# Autodesk Inventor assembly: WheelAssembly
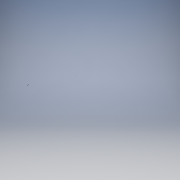
[picture p0: Inventor's stored thumbnail of the model, 180x180]
Saved by Autodesk Inventor 2016 (Build 200138000, 138)
## iProperties
Created: 2016-09-10
Part Number: WheelAssembly
Document SubType Name: Assembly
Designer: RoboticsUser
Author: RoboticsUser
## Documents named in this file (10)
- C:\Robotics\2016-17_CAD\WheelAssembly.iam
- C:\Robotics\CAD\2015-16\custom cad parts\am-2648_4inWheel8mmHub.ipt
- C:\Robotics\CAD\2015-16\COTSParts\Actobotics\545 parts\545556.ipt
- C:\Robotics\CAD\2015-16\COTSParts\Actobotics\615 parts\615102.ipt
- C:\Robotics\CAD\2015-16\COTSParts\Actobotics\634 parts\634080.ipt
- C:\Users\RoboticsUser\Desktop\2015-16 CAD\COTSParts\Actobotics\555 parts\555176.ipt
- C:\Users\RoboticsUser\Desktop\2015-16 CAD\COTSParts\Actobotics\am-2964NeveRest.ipt
- C:\Users\RoboticsUser\Desktop\2015-16 CAD\COTSParts\Actobotics\585 parts\585462.ipt
- C:\Users\RoboticsUser\Desktop\2015-16 CAD\COTSParts\Actobotics\615 parts\615114.ipt
- C:\Users\RoboticsUser\Desktop\2015-16 CAD\COTSParts\Actobotics\585 parts\585454.ipt
## Components (22 placed, 9 different names)
1. 545556:5 — Insert:10, Insert:11
2. am-2648_4inWheel8mmHub:2 — Insert:2, Insert:10
3. 545556:2 — Insert:2, Insert:9
4. 634080:1
5. 615102:3
6. 615102:4 — Insert:11
7. 634080:2 — Insert:9, Insert:24
8. am-2648_4inWheel8mmHub:3
9. 545556:6
10. 615102:5
11. 545556:7
12. 634080:3 — Insert:25
13. 555176:2 — Insert:17
14. am-2964NeveRest:2 — Insert:17, Insert:23
15. 545556:8 — Insert:19, Insert:23
16. 615114:2 — Insert:19
17. 615114:3 — Insert:18
18. 545556:9 — Insert:18, Insert:26
19. 555176:3 — Insert:22, Insert:27, Insert:28
20. am-2964NeveRest:3 — Insert:22, Insert:26
21. 585462:1 — Insert:24, Insert:25, Mate:1, Flush:4, Flush:5
22. 585454:2 — Mate:1, Flush:4, Flush:5, Insert:27, Insert:28
## Relationships (21: Insert 18, Flush 2, Mate 1)
- Insert:2: am-2648_4inWheel8mmHub:2 ↔ 545556:2
- Insert:9 (-12.7 mm): 545556:2 ↔ 634080:2
- Insert:10 (3.175 mm): 545556:5 ↔ am-2648_4inWheel8mmHub:2
- Insert:11 (2.54 mm): 545556:5 ↔ 615102:4
- [Insert]: am-2648_4inWheel8mmHub:3 ↔ 545556:6
- [Insert] (-12.7 mm): 545556:6 ↔ 634080:3
- [Insert] (3.175 mm): am-2648_4inWheel8mmHub:3 ↔ 545556:7
- [Insert] (2.54 mm): 615102:5 ↔ 545556:7
- Insert:17: 555176:2 ↔ am-2964NeveRest:2
- Insert:18: 615114:3 ↔ 545556:9
- Insert:19: 545556:8 ↔ 615114:2
- Insert:22: 555176:3 ↔ am-2964NeveRest:3
- Insert:23: am-2964NeveRest:2 ↔ 545556:8
- Insert:24 (25.4 mm): 634080:2 ↔ 585462:1
- Insert:25: 634080:3 ↔ 585462:1
- Insert:26: 545556:9 ↔ am-2964NeveRest:3
- Mate:1: 585462:1 ↔ 585454:2
- Flush:4 (19.05 mm): 585462:1 ↔ 585454:2
- Flush:5 (-76.2 mm): 585462:1 ↔ 585454:2
- Insert:27: 555176:3 ↔ 585454:2
- Insert:28: 555176:3 ↔ 585454:2
## Named parameters: d32_d31 = 2.54 mm, d33_d17 = 0 mm, d34_d28 = -12.7 mm, d35_d29 = 3.175 mm
